# Autodesk Inventor assembly: Connecting Rod
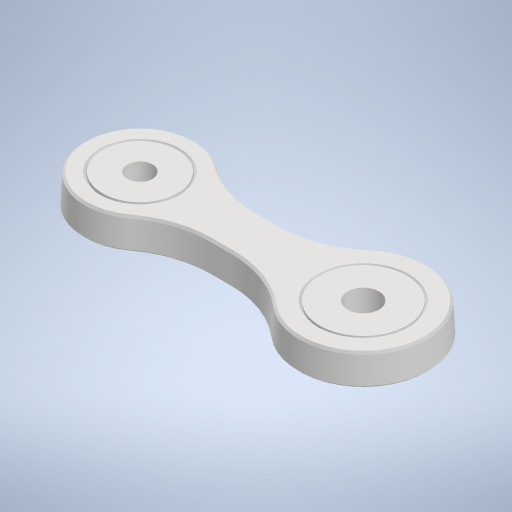
[picture p0: Inventor's stored thumbnail of the model, 512x512]
Saved by Autodesk Inventor 2023 (Build 270158000, 158)
## iProperties
Created: 2022-12-22
Part Number: Connecting Rod
Document SubType Name: Assembly
Designer: tgr41
Author: tgr41
## Documents named in this file (4)
- C:\Users\tgr41\OneDrive\Documents\Repositories\Steam-Engine\2 Inch V3\Connecting Rod.iam
- C:\Users\tgr41\OneDrive\Documents\Repositories\Steam-Engine\2 Inch V3\Connecting Rod.ipt
- C:\Users\tgr41\OneDrive\Documents\Repositories\Steam-Engine\2 Inch V3\Wrist Pin Bearing.ipt
- C:\Users\tgr41\OneDrive\Documents\Repositories\Steam-Engine\2 Inch V3\Connecting Rod Bearing.ipt
## Components (3 placed, 3 different names)
1. Connecting Rod:1 — Mate:1, Mate:2, Flush:1, Flush:2
2. Wrist Pin Bearing:1 — Mate:2, Flush:1
3. Connecting Rod Bearing:1 — Mate:1, Flush:2
## Relationships (4: Mate 2, Flush 2)
- Mate:1: Connecting Rod:1 ↔ Connecting Rod Bearing:1
- Mate:2: Connecting Rod:1 ↔ Wrist Pin Bearing:1
- Flush:1: Connecting Rod:1 ↔ Wrist Pin Bearing:1
- Flush:2: Connecting Rod:1 ↔ Connecting Rod Bearing:1
